# Autodesk Inventor assembly: 652-19
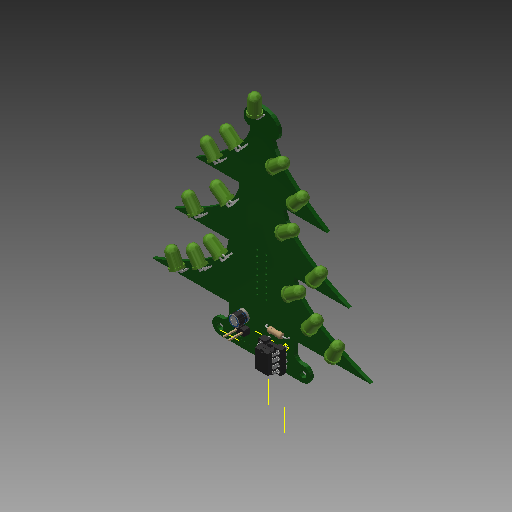
[picture p0: Inventor's stored thumbnail of the model, 512x512]
Saved by Autodesk Inventor 2018.3 (Build 223284000, 284)
## iProperties
Company: UNH Makerspace
Created: 2019-07-26
Part Number: 652-19
Document SubType Name: Assembly
Designer: Electro707
Engineer: Jamal Bouajjaj
Author: Electro707
Title: Dual Construction Tree - Mounting Holes
Revision Number: N/A
## iProperties of the stored document PCB.iam
Created: 2019-12-02
Part Number: PCB
Description: KiCad electronic assembly
Document SubType Name: Assembly
Designer: Electro707
Authority: Unknown
Company: A Company
Sending System: KiCad to STEP converter
Preprocessor: Open CASCADE STEP processor 6.9
Title: PCB.step
Author: An Author
## iProperties of the stored document CP_Radial_D5.0mm_P2.50mm.iam
Created: 2019-07-26
Part Number: CP_Radial_D5.0mm_P2.50mm
Document SubType Name: Assembly
Designer: Electro707
Author: Electro707
## iProperties of the stored document SOLID_5.ipt
Created: 2019-07-26
Part Number: SOLID_5
Material: Generic
Document SubType Name: Modeling
Designer: Electro707
Density: 1 g/cm^3
Appearance: Default
Mass: 0.20853 g
Surface Area: 4.37731 cm^2
Volume: 0.20853 cm^3
Author: Electro707
## iProperties of the stored document SOLID.ipt
Created: 2019-07-26
Part Number: SOLID
Material: Generic
Document SubType Name: Modeling
Designer: Electro707
Density: 1 g/cm^3
Appearance: Default
Author: Electro707
## iProperties of the stored document SOIC-16_3.9x9.9mm_P1.27mm.iam
Created: 2019-07-26
Part Number: SOIC-16_3.9x9.9mm_P1.27mm
Document SubType Name: Assembly
Designer: Electro707
Author: Electro707
## iProperties of the stored document SOLID_2.ipt
Created: 2019-07-26
Part Number: SOLID_2
Material: Generic
Document SubType Name: Modeling
Designer: Electro707
Density: 1 g/cm^3
Appearance: Default
Author: Electro707
## iProperties of the stored document PinHeader_1x02_P2.54mm_Vertical.iam
Created: 2019-07-26
Part Number: PinHeader_1x02_P2.54mm_Vertical
Document SubType Name: Assembly
Designer: Electro707
Author: Electro707
## iProperties of the stored document SOLID_1.ipt
Created: 2019-07-26
Part Number: SOLID_1
Material: Generic
Document SubType Name: Modeling
Designer: Electro707
Density: 1 g/cm^3
Appearance: Default
Author: Electro707
## iProperties of the stored document LED_D5.0mm_Horizontal_O1.27mm_Z3.0mm.iam
Created: 2019-07-26
Part Number: LED_D5.0mm_Horizontal_O1.27mm_Z3.0mm
Document SubType Name: Assembly
Designer: Electro707
Author: Electro707
## iProperties of the stored document C_1206_3216Metric.iam
Created: 2019-11-06
Part Number: C_1206_3216Metric
Document SubType Name: Assembly
Designer: Electro707
Author: Electro707
## iProperties of the stored document SOLID_6.ipt
Created: 2019-07-26
Part Number: SOLID_6
Material: Generic
Document SubType Name: Modeling
Designer: Electro707
Density: 1 g/cm^3
Appearance: Default
Mass: 0.0300937 g
Surface Area: 0.759695 cm^2
Volume: 0.0300937 cm^3
Author: Electro707
## iProperties of the stored document COMPOUND.ipt
Created: 2019-07-26
Part Number: COMPOUND
Material: Generic
Document SubType Name: Modeling
Designer: Electro707
Density: 1 g/cm^3
Appearance: Default
Author: Electro707
## iProperties of the stored document SOLID.ipt
Created: 2019-11-06
Part Number: SOLID
Material: Generic
Document SubType Name: Modeling
Designer: Electro707
Density: 1 g/cm^3
Appearance: Default
Mass: 0.0929769 g
Surface Area: 1.47718 cm^2
Volume: 0.0929769 cm^3
Author: Electro707
## iProperties of the stored document SOLID_4.ipt
Created: 2019-07-26
Part Number: SOLID_4
Material: Generic
Document SubType Name: Modeling
Designer: Electro707
Density: 1 g/cm^3
Appearance: Default
Author: Electro707
## iProperties of the stored document R_1206_3216Metric.iam
Created: 2019-11-06
Part Number: R_1206_3216Metric
Document SubType Name: Assembly
Designer: Electro707
Author: Electro707
## iProperties of the stored document R_Axial_DIN0207_L6.3mm_D2.5mm_P10.16mm_Horizontal.iam
Created: 2019-07-26
Part Number: R_Axial_DIN0207_L6.3mm_D2.5mm_P10.16mm_Horizontal
Document SubType Name: Assembly
Designer: Electro707
Author: Electro707
## iProperties of the stored document DIP-8_W7.62mm_Socket.iam
Created: 2019-07-26
Part Number: DIP-8_W7.62mm_Socket
Document SubType Name: Assembly
Designer: Electro707
Author: Electro707
## iProperties of the stored document SOLID_3.ipt
Created: 2019-07-26
Part Number: SOLID_3
Material: Generic
Document SubType Name: Modeling
Designer: Electro707
Density: 1 g/cm^3
Appearance: Default
Mass: 0.0393822 g
Surface Area: 1.08508 cm^2
Volume: 0.0393822 cm^3
Author: Electro707
## Documents named in this file (22)
- **F:\Projects\UNH MakerSpace Kits\2019 - Winter Holiday\Dual Tree Construction\CAD-Inventor\Assembly - Main Tree.iam*LocalDocs*xG0zgcc3sLp4ruqobEclatnt14b*PCB.iam
- **F:\Projects\UNH MakerSpace Kits\2019 - Winter Holiday\Dual Tree Construction\CAD-Inventor\Assembly - Main Tree.iam*LocalDocs*xFbs23fwjPixpuo4gO4eu3sutGb*PinHeader_1x02_P2.54mm_Vertical.iam
- **F:\Projects\UNH MakerSpace Kits\2019 - Winter Holiday\Dual Tree Construction\CAD-Inventor\Assembly - Main Tree.iam*LocalDocs*xNlbxmcraAyepelgmCbfopdmo2c*LED_D5.0mm_Horizontal_O1.27mm_Z3.0mm.iam
- **F:\Projects\UNH MakerSpace Kits\2019 - Winter Holiday\Dual Tree Construction\CAD-Inventor\Assembly - Main Tree.iam*LocalDocs*x3pdi2fncTeuhuv0l1kkyy1puDh*SOIC-16_3.9x9.9mm_P1.27mm.iam
- **F:\Projects\UNH MakerSpace Kits\2019 - Winter Holiday\Dual Tree Construction\CAD-Inventor\Assembly - Main Tree.iam*LocalDocs*xYrxouptqOupyutw5Ui0ymssb0h*DIP-8_W7.62mm_Socket.iam
- **F:\Projects\UNH MakerSpace Kits\2019 - Winter Holiday\Dual Tree Construction\CAD-Inventor\Assembly - Main Tree.iam*LocalDocs*xSynj4mbaYi11ewctZ5fxp2bl3e*R_Axial_DIN0207_L6.3mm_D2.5mm_P10.16mm_Horizontal.iam
- **F:\Projects\UNH MakerSpace Kits\2019 - Winter Holiday\Dual Tree Construction\CAD-Inventor\Assembly - Main Tree.iam*LocalDocs*xE1ocay3dQ0aweg03Hx1l4ram4d*CP_Radial_D5.0mm_P2.50mm.iam
- **F:\Projects\UNH MakerSpace Kits\2019 - Winter Holiday\Dual Tree Construction\CAD-Inventor\Assembly - Main Tree.iam*LocalDocs*xMkoztgkfWk1lelovS4pxxtneWc*COMPOUND.ipt
- **F:\Projects\UNH MakerSpace Kits\2019 - Winter Holiday\Dual Tree Construction\CAD-Inventor\Assembly - Main Tree.iam*LocalDocs*xIb1xkek2Yxerut0wZrszpwszEf*C_1206_3216Metric.iam
- **F:\Projects\UNH MakerSpace Kits\2019 - Winter Holiday\Dual Tree Construction\CAD-Inventor\Assembly - Main Tree.iam*LocalDocs*xTjflrd1eZia2es4nRdrxknfeZf*R_1206_3216Metric.iam
- **F:\Projects\UNH MakerSpace Kits\2019 - Winter Holiday\Dual Tree Construction\CAD-Inventor\Assembly - Main Tree.iam*LocalDocs*xRivwwja4G2gyuxklMlmmyjlr5f*SOLID.ipt
- **F:\Projects\UNH MakerSpace Kits\2019 - Winter Holiday\Dual Tree Construction\CAD-Inventor\Assembly - Main Tree.iam*LocalDocs*x3izbotpcBwxvehgiV0ok1uq2Md*SOLID_5.ipt
- **F:\Projects\UNH MakerSpace Kits\2019 - Winter Holiday\Dual Tree Construction\CAD-Inventor\Assembly - Main Tree.iam*LocalDocs*x0jb5n1hx2uzve50y0pqkgnmtWf*SOLID.ipt
- **F:\Projects\UNH MakerSpace Kits\2019 - Winter Holiday\Dual Tree Construction\CAD-Inventor\Assembly - Main Tree.iam*LocalDocs*xO5bpx2d200gqur0wO5vjfjgs2f*SOLID_4.ipt
- **F:\Projects\UNH MakerSpace Kits\2019 - Winter Holiday\Dual Tree Construction\CAD-Inventor\Assembly - Main Tree.iam*LocalDocs*xFdv5ifzqAaflenowFh1febphPe*SOLID_2.ipt
- **F:\Projects\UNH MakerSpace Kits\2019 - Winter Holiday\Dual Tree Construction\CAD-Inventor\Assembly - Main Tree.iam*LocalDocs*xYzys2aoqQ4jjeacn1czxhvrwVd*SOLID_3.ipt
- **F:\Projects\UNH MakerSpace Kits\2019 - Winter Holiday\Dual Tree Construction\CAD-Inventor\Assembly - Main Tree.iam*LocalDocs*xFtxalom4Vfg5etcxJkotdhvzHe*SOLID_1.ipt
- **F:\Projects\UNH MakerSpace Kits\2019 - Winter Holiday\Dual Tree Construction\CAD-Inventor\Assembly - Main Tree.iam*LocalDocs*xG5y41pfo2qaluwwgRv3gbdkqCa*SOLID_6.ipt
- F:\Projects\UNH MakerSpace Kits\2019 - Winter Holiday\Dual Tree Construction\GitHub Folder\CAD - Inventor\Assembly - Main Tree.iam
- **F:\Projects\UNH MakerSpace Kits\2019 - Winter Holiday\Dual Tree Construction\GitHub Folder\CAD - Inventor\Assembly - Main Tree.iam*LocalDocs*xG0zgcc3sLp4ruqobEclatnt14b*PCB.iam
- F:\Projects\UNH MakerSpace Kits\2019 - Winter Holiday\Dual Tree Construction\GitHub Folder\CAD - Inventor\DIP-8_W7.62mm.ipt
- F:\Projects\UNH MakerSpace Kits\2019 - Winter Holiday\Dual Tree Construction\GitHub Folder\CAD - Inventor\Main Tree.step
## Components (2 placed, 2 different names)
1. PCB:1 [sub-assembly] — Mate:13, Mate:14, Mate:15
2. DIP-8_W7.62mm:1 — Mate:1, Mate:2, Mate:3, Mate:4, Mate:7, Mate:8, Mate:9, Mate:10, Mate:14
## Relationships (15: Mate 15)
- Mate:1: DIP-8_W7.62mm:1
- Mate:2: DIP-8_W7.62mm:1
- Mate:3: DIP-8_W7.62mm:1
- Mate:4: DIP-8_W7.62mm:1
- Mate:5
- Mate:6
- Mate:7: DIP-8_W7.62mm:1
- Mate:8: DIP-8_W7.62mm:1
- Mate:9: DIP-8_W7.62mm:1
- Mate:10: DIP-8_W7.62mm:1
- Mate:11
- Mate:12
- Mate:13: PCB:1
- Mate:14: PCB:1 ↔ DIP-8_W7.62mm:1
- Mate:15: PCB:1
